# Autodesk Inventor assembly: standing_robot_ver.1
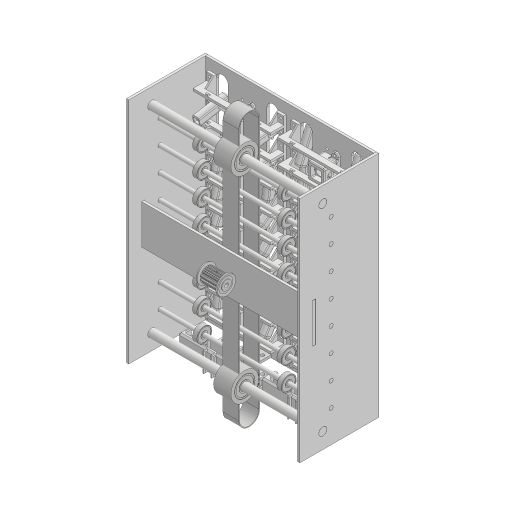
[picture p0: Inventor's stored thumbnail of the model, 512x512]
Saved by Autodesk Inventor 2024 (Build 280153000, 153)
## iProperties
Created: 2023-11-09
Part Number: standing_robot_ver.1
Document SubType Name: Assembly
Designer: moonshot
Author: moonshot
## Documents named in this file (18)
- C:\Users\moonshot\Desktop\ikisawa\ikisawa\experiment8_standing\standing_robot\standing_robot_ver.4.iam
- C:\Users\moonshot\Desktop\ikisawa\ikisawa\experiment8_standing\leg_unit\cover.ver1.ipt
- C:\Users\moonshot\Desktop\ikisawa\ikisawa\experiment8_standing\leg_unit\leg.ipt
- C:\Users\moonshot\Desktop\ikisawa\ikisawa\experiment8_standing\leg_unit\shaft_leg.ipt
- C:\Users\moonshot\Desktop\ikisawa\ikisawa\experiment8_standing\leg_unit\parent_ver.1.ipt
- C:\Users\moonshot\Desktop\ikisawa\ikisawa\experiment8_standing\floor\floor_ver.1.ipt
- C:\Users\moonshot\Desktop\ikisawa\ikisawa\experiment8_standing\belt\ATBT-720T5200-B-P30_info-1-16-16.ipt
- C:\Users\moonshot\Desktop\ikisawa\ikisawa\experiment8_standing\guide\guide_ver.2.ipt
- C:\Users\moonshot\Desktop\ikisawa\ikisawa\experiment8_standing\pulley\AIS2024\TTPS12T5200-A-P5.iam
- C:\Users\moonshot\Desktop\ikisawa\ikisawa\experiment8_standing\adapter\adapter_repulsive_force_ver.3.ipt
- C:\Users\moonshot\Desktop\ikisawa\ikisawa\experiment8_standing\wall\wall_ver.1.ipt
- C:\Users\moonshot\Desktop\ikisawa\ikisawa\experiment8_standing\bearing\C-SE635ZZ.ipt
- C:\Users\moonshot\Desktop\ikisawa\ikisawa\experiment8_standing\bearing\shaft_bearing\shaft_bearing.ipt
- C:\Users\moonshot\Desktop\ikisawa\ikisawa\experiment8_standing\stage\stage_ver.1.ipt
- C:\Users\moonshot\Desktop\ikisawa\ikisawa\experiment8_standing\idler\AIS2024\C-AFBD22-35W.iam
- C:\Users\moonshot\Desktop\ikisawa\ikisawa\experiment8_standing\bearing\shaft_bearing\shaft_idler_ver.1.ipt
- C:\Users\moonshot\Desktop\ikisawa\ikisawa\experiment8_standing\magnet\magnet_10-10-6.ipt
- C:\Users\moonshot\Desktop\ikisawa\ikisawa\experiment8_standing\magnet\magnet_holder_ver.1.ipt
## Components (146 placed, 17 different names)
1. floor_ver.1:1 — フラッシュ:3, フラッシュ:4, フラッシュ:5, メイト:8, メイト:9, メイト:10, メイト:16, メイト:17, メイト:18, メイト:4, メイト:5, メイト:15, メイト:14, メイト:19, メイト:20, メイト:21, メイト:40, フラッシュ:11, フラッシュ:12, メイト:55, メイト:56, メイト:60, メイト:61, メイト:62, メイト:63, メイト:67, メイト:68, メイト:69, メイト:70, メイト:71, メイト:72, メイト:73, メイト:74, メイト:75, メイト:79, メイト:80, メイト:81, メイト:82, メイト:83, メイト:87, メイト:88, メイト:89, メイト:90, メイト:91, メイト:95, メイト:96, メイト:97, メイト:98, メイト:99, メイト:103, メイト:104, メイト:105, メイト:106, メイト:107, メイト:111, メイト:112, メイト:113, メイト:114, メイト:115, メイト:119, メイト:120, メイト:121, メイト:122, メイト:123, メイト:127, メイト:128, メイト:129, メイト:130, メイト:131, メイト:135, メイト:136, メイト:137, メイト:138, メイト:139, メイト:143, メイト:144, メイト:145, メイト:146, メイト:147, メイト:151, メイト:152, メイト:153, メイト:154, メイト:155, メイト:159, メイト:160, メイト:161, メイト:162, メイト:163, メイト:164, メイト:165, メイト:166, メイト:167, メイト:168, メイト:169, メイト:170, メイト:171, メイト:172, メイト:173, メイト:174, メイト:175, メイト:176, メイト:177, メイト:178, メイト:179, メイト:180, メイト:181, メイト:182, メイト:183, メイト:184, メイト:185, メイト:186, メイト:187, メイト:188, メイト:189, メイト:190, メイト:191, メイト:192, メイト:193, メイト:194, メイト:195, メイト:196, メイト:197, メイト:198, メイト:199, メイト:200, メイト:201, メイト:202, メイト:203, メイト:204, メイト:205, メイト:206, メイト:207, メイト:208, メイト:209, メイト:210, メイト:211, メイト:212, メイト:213, メイト:214, メイト:255, フラッシュ:51, フラッシュ:52
2. ATBT-720T5200-B-P30_info-1-16-16:1 — メイト:6, フラッシュ:6, メイト:32, メイト:33, メイト:34, メイト:35
3. TTPS12T5200-A-P5:1 [sub-assembly] — メイト:29, フラッシュ:9, メイト:50
4. adapter_repulsive_force_ver.3:1 — メイト:30, メイト:31, メイト:32, メイト:33, メイト:34, メイト:36, メイト:268, フラッシュ:59, フラッシュ:60, メイト:269, メイト:270, フラッシュ:61, メイト:275, メイト:276
5. adapter_repulsive_force_ver.3:2 — メイト:30, メイト:31, メイト:35, メイト:271, フラッシュ:62, メイト:272, メイト:273, フラッシュ:63, メイト:274, フラッシュ:64, フラッシュ:65, メイト:277, メイト:278
6. wall_ver.1:2 — メイト:40, フラッシュ:11, フラッシュ:12, フラッシュ:13, メイト:46, フラッシュ:14, メイト:48, メイト:51, フラッシュ:43, メイト:217, フラッシュ:44, メイト:218, フラッシュ:45, メイト:219, フラッシュ:46, メイト:220, フラッシュ:47, メイト:221, メイト:222, メイト:223, フラッシュ:48, フラッシュ:49, フラッシュ:50, メイト:252
7. stage_ver.1:1 — メイト:44, メイト:45, メイト:50, メイト:51
8. C-AFBD22-35W:1 [sub-assembly] — メイト:47, メイト:49
9. shaft_idler_ver.1:1 — フラッシュ:14, メイト:48, メイト:49
10. shaft_idler_ver.1:2 — フラッシュ:50, メイト:252, メイト:254
11. C-AFBD22-35W:2 [sub-assembly] — メイト:253, メイト:254
12. wall_ver.1:3 — メイト:255, フラッシュ:51, フラッシュ:52
13. magnet_10-10-6:1 — メイト:256, メイト:257, フラッシュ:53, メイト:268, フラッシュ:59, メイト:275
14. magnet_10-10-6:2 — メイト:258, メイト:259, フラッシュ:54, メイト:269, メイト:276
15. magnet_10-10-6:3 — メイト:260, メイト:261, フラッシュ:55, メイト:270, フラッシュ:61
16. magnet_10-10-6:4 — メイト:262, メイト:263, フラッシュ:56, メイト:271, メイト:272, フラッシュ:65
17. magnet_10-10-6:5 — メイト:266, メイト:267, フラッシュ:58, メイト:274, メイト:277
18. magnet_10-10-6:6 — メイト:264, メイト:265, フラッシュ:57, メイト:273, メイト:278
19. magnet_holder_ver.1:1 — メイト:256, メイト:257, フラッシュ:53
20. magnet_holder_ver.1:2 — メイト:258, メイト:259, フラッシュ:54, フラッシュ:60
21. magnet_holder_ver.1:3 — メイト:260, メイト:261, フラッシュ:55
22. magnet_holder_ver.1:4 — メイト:262, メイト:263, フラッシュ:56, フラッシュ:62
23. magnet_holder_ver.1:5 — メイト:264, メイト:265, フラッシュ:57, フラッシュ:63
24. magnet_holder_ver.1:6 — メイト:266, メイト:267, フラッシュ:58, フラッシュ:64
25. cover.ver1:1 — フラッシュ:1, スライダ:1, メイト:8, メイト:9, メイト:10, メイト:36
26. leg:1 — メイト:2, メイト:5
27. leg:2 — メイト:3, メイト:4
28. shaft_leg:1 — メイト:1, フラッシュ:2, メイト:2, メイト:3
29. parent_ver.1:1 — フラッシュ:1, スライダ:1, メイト:1, フラッシュ:2, メイト:41
30. cover.ver1:2 — メイト:16, メイト:17, メイト:18
31. leg:3 — メイト:15, メイト:71
32. leg:4 — メイト:14
33. shaft_leg:2
34. parent_ver.1:2 — メイト:225
35. cover.ver1:3 — メイト:55, メイト:56, メイト:63
36. leg:5
37. leg:6 — メイト:70
38. shaft_leg:3
39. parent_ver.1:3 — メイト:231
40. cover.ver1:4 — メイト:60, メイト:61, メイト:62
41. leg:7 — メイト:73
42. leg:8 — メイト:72
43. shaft_leg:4
44. parent_ver.1:4 — メイト:234
45. cover.ver1:5 — メイト:67, メイト:68, メイト:69
46. leg:9 — メイト:74
47. leg:10 — メイト:75
48. shaft_leg:5
49. parent_ver.1:5 — メイト:239
50. cover.ver1:6 — メイト:79, メイト:80, メイト:81
51. leg:11 — メイト:83
52. leg:12 — メイト:82
53. shaft_leg:6
54. parent_ver.1:6 — メイト:243
55. cover.ver1:7 — メイト:87, メイト:88, メイト:89
56. leg:13 — メイト:90
57. leg:14 — メイト:91
58. shaft_leg:7
59. parent_ver.1:7 — メイト:247
60. cover.ver1:8 — メイト:95, メイト:96, メイト:97
61. leg:15 — メイト:98
62. leg:16 — メイト:99
63. shaft_leg:8
64. parent_ver.1:8 — メイト:251
65. cover.ver1:9 — メイト:103, メイト:104, メイト:105, メイト:216
66. leg:17 — メイト:106
67. leg:18 — メイト:107
68. shaft_leg:9
69. parent_ver.1:9
70. cover.ver1:10 — メイト:111, メイト:112, メイト:113
71. leg:19 — メイト:114
72. leg:20 — メイト:115
73. shaft_leg:10
74. parent_ver.1:10 — メイト:230
75. cover.ver1:11 — メイト:119, メイト:120, メイト:121
76. leg:21 — メイト:123
77. leg:22 — メイト:122
78. shaft_leg:11
79. parent_ver.1:11 — メイト:227
80. cover.ver1:12 — メイト:127, メイト:128, メイト:129
81. leg:23 — メイト:131
82. leg:24 — メイト:130
83. shaft_leg:12
84. parent_ver.1:12 — メイト:235
85. cover.ver1:13 — メイト:135, メイト:136, メイト:137
86. leg:25 — メイト:139
87. leg:26 — メイト:138
88. shaft_leg:13
89. parent_ver.1:13 — メイト:238
90. cover.ver1:14 — メイト:143, メイト:144, メイト:145
91. leg:27 — メイト:147
92. leg:28 — メイト:146
93. shaft_leg:14
94. parent_ver.1:14 — メイト:242
95. cover.ver1:15 — メイト:151, メイト:152, メイト:153
96. leg:29 — メイト:154
97. leg:30 — メイト:155
98. shaft_leg:15
99. parent_ver.1:15 — メイト:246
100. cover.ver1:16 — メイト:159, メイト:160, メイト:161
101. leg:31 — メイト:163
102. leg:32 — メイト:162
103. shaft_leg:16
104. parent_ver.1:16 — メイト:250
105. guide_ver.2:1 — メイト:19, メイト:20, メイト:21
106. guide_ver.2:2 — メイト:164, メイト:165, メイト:166
107. guide_ver.2:3 — メイト:167, メイト:168, メイト:169
108. guide_ver.2:4 — メイト:170, メイト:171, メイト:172
109. guide_ver.2:5 — メイト:173, メイト:174, メイト:175
110. guide_ver.2:6 — メイト:176, メイト:177, メイト:178
111. guide_ver.2:7 — メイト:179, メイト:180, メイト:181
112. guide_ver.2:8 — メイト:182, メイト:183, メイト:184
113. guide_ver.2:9 — メイト:185, メイト:186, メイト:187
114. guide_ver.2:10 — メイト:188, メイト:189, メイト:190
115. guide_ver.2:11 — メイト:191, メイト:192, メイト:193
116. guide_ver.2:12 — メイト:194, メイト:195, メイト:196
117. guide_ver.2:13 — メイト:197, メイト:198, メイト:199
118. guide_ver.2:14 — メイト:200, メイト:201, メイト:202
119. guide_ver.2:15 — メイト:203, メイト:204, メイト:205
120. guide_ver.2:16 — メイト:206, メイト:207, メイト:208
121. guide_ver.2:17 — メイト:209, メイト:210, メイト:211
122. guide_ver.2:18 — メイト:212, メイト:213, メイト:214
123. shaft_bearing:1 — フラッシュ:13, メイト:43, メイト:46, メイト:215
124. shaft_bearing:2 — フラッシュ:43, メイト:217, メイト:224, メイト:226
125. shaft_bearing:3 — フラッシュ:44, メイト:218, メイト:228, メイト:229
126. shaft_bearing:4 — フラッシュ:45, メイト:219, メイト:232, メイト:233
127. shaft_bearing:5 — フラッシュ:46, メイト:220, メイト:236, メイト:237
128. shaft_bearing:6 — フラッシュ:47, メイト:221, メイト:240, メイト:241
129. shaft_bearing:7 — メイト:222, フラッシュ:48, メイト:244, メイト:245
130. shaft_bearing:8 — メイト:223, フラッシュ:49, メイト:248, メイト:249
131. C-SE635ZZ:1 — メイト:41, メイト:43
132. C-SE635ZZ:2 — メイト:215, メイト:216
133. C-SE635ZZ:3 — メイト:224, メイト:225
134. C-SE635ZZ:4 — メイト:226, メイト:227
135. C-SE635ZZ:5 — メイト:228, メイト:231
136. C-SE635ZZ:6 — メイト:229, メイト:230
137. C-SE635ZZ:7 — メイト:232, メイト:234
138. C-SE635ZZ:8 — メイト:233, メイト:235
139. C-SE635ZZ:9 — メイト:236, メイト:239
140. C-SE635ZZ:10 — メイト:237, メイト:238
141. C-SE635ZZ:11 — メイト:240, メイト:243
142. C-SE635ZZ:12 — メイト:241, メイト:242
143. C-SE635ZZ:13 — メイト:244, メイト:247
144. C-SE635ZZ:14 — メイト:245, メイト:246
145. C-SE635ZZ:15 — メイト:248, メイト:251
146. C-SE635ZZ:16 — メイト:249, メイト:250
## Relationships (346: Mate 266, Flush 64, TranslationJoint 16)
- フラッシュ:1 [Flush]: cover.ver1:1 ↔ parent_ver.1:1
- スライダ:1 [TranslationJoint]: cover.ver1:1 ↔ parent_ver.1:1
- メイト:1 [Mate]: shaft_leg:1 ↔ parent_ver.1:1
- フラッシュ:2 [Flush]: shaft_leg:1 ↔ parent_ver.1:1
- メイト:2 [Mate]: leg:1 ↔ shaft_leg:1
- メイト:3 [Mate]: leg:2 ↔ shaft_leg:1
- メイト:4 [Mate] (2.5 mm): floor_ver.1:1 ↔ leg:2
- メイト:5 [Mate] (2.5 mm): floor_ver.1:1 ↔ leg:1
- フラッシュ:3 [Flush]: floor_ver.1:1
- フラッシュ:4 [Flush]: floor_ver.1:1
- フラッシュ:5 [Flush]: floor_ver.1:1
- メイト:6 [Mate]: ATBT-720T5200-B-P30_info-1-16-16:1
- フラッシュ:6 [Flush]: ATBT-720T5200-B-P30_info-1-16-16:1
- メイト:8 [Mate]: floor_ver.1:1 ↔ cover.ver1:1
- メイト:9 [Mate]: floor_ver.1:1 ↔ cover.ver1:1
- メイト:10 [Mate]: floor_ver.1:1 ↔ cover.ver1:1
- [Flush]: cover.ver1:2 ↔ parent_ver.1:2
- [TranslationJoint]: cover.ver1:2 ↔ parent_ver.1:2
- [Mate]: shaft_leg:2 ↔ parent_ver.1:2
- [Flush]: shaft_leg:2 ↔ parent_ver.1:2
- [Mate]: leg:3 ↔ shaft_leg:2
- [Mate]: leg:4 ↔ shaft_leg:2
- メイト:14 [Mate] (2.5 mm): floor_ver.1:1 ↔ leg:4
- メイト:15 [Mate] (2.5 mm): floor_ver.1:1 ↔ leg:3
- メイト:16 [Mate]: floor_ver.1:1 ↔ cover.ver1:2
- メイト:17 [Mate]: floor_ver.1:1 ↔ cover.ver1:2
- メイト:18 [Mate]: floor_ver.1:1 ↔ cover.ver1:2
- メイト:19 [Mate]: floor_ver.1:1 ↔ guide_ver.2:1
- メイト:20 [Mate]: floor_ver.1:1 ↔ guide_ver.2:1
- メイト:21 [Mate]: floor_ver.1:1 ↔ guide_ver.2:1
- メイト:29 [Mate]: TTPS12T5200-A-P5:1
- フラッシュ:9 [Flush]: TTPS12T5200-A-P5:1
- メイト:50 [Mate] (13 mm): TTPS12T5200-A-P5:1 ↔ stage_ver.1:1
- メイト:30 [Mate]: adapter_repulsive_force_ver.3:1 ↔ adapter_repulsive_force_ver.3:2
- メイト:31 [Mate]: adapter_repulsive_force_ver.3:1 ↔ adapter_repulsive_force_ver.3:2
- メイト:32 [Mate]: ATBT-720T5200-B-P30_info-1-16-16:1 ↔ adapter_repulsive_force_ver.3:1
- メイト:33 [Mate]: ATBT-720T5200-B-P30_info-1-16-16:1 ↔ adapter_repulsive_force_ver.3:1
- メイト:34 [Mate]: ATBT-720T5200-B-P30_info-1-16-16:1 ↔ adapter_repulsive_force_ver.3:1
- メイト:35 [Mate]: ATBT-720T5200-B-P30_info-1-16-16:1 ↔ adapter_repulsive_force_ver.3:2
- メイト:36 [Mate] (1 mm): adapter_repulsive_force_ver.3:1 ↔ cover.ver1:1
- メイト:40 [Mate]: floor_ver.1:1 ↔ wall_ver.1:2
- フラッシュ:11 [Flush]: floor_ver.1:1 ↔ wall_ver.1:2
- フラッシュ:12 [Flush]: floor_ver.1:1 ↔ wall_ver.1:2
- メイト:41 [Mate]: parent_ver.1:1 ↔ C-SE635ZZ:1
- フラッシュ:13 [Flush]: wall_ver.1:2 ↔ shaft_bearing:1
- メイト:43 [Mate]: shaft_bearing:1 ↔ C-SE635ZZ:1
- メイト:44 [Mate]: stage_ver.1:1
- メイト:45 [Mate]: stage_ver.1:1
- メイト:46 [Mate]: wall_ver.1:2 ↔ shaft_bearing:1
- メイト:47 [Mate]: C-AFBD22-35W:1
- フラッシュ:14 [Flush]: wall_ver.1:2 ↔ shaft_idler_ver.1:1
- メイト:48 [Mate]: wall_ver.1:2 ↔ shaft_idler_ver.1:1
- メイト:49 [Mate]: C-AFBD22-35W:1 ↔ shaft_idler_ver.1:1
- メイト:51 [Mate] (20 mm): wall_ver.1:2 ↔ stage_ver.1:1
- [Flush]: cover.ver1:3 ↔ parent_ver.1:3
- [TranslationJoint]: cover.ver1:3 ↔ parent_ver.1:3
- [Mate]: shaft_leg:3 ↔ parent_ver.1:3
- [Flush]: shaft_leg:3 ↔ parent_ver.1:3
- [Mate]: leg:5 ↔ shaft_leg:3
- [Mate]: leg:6 ↔ shaft_leg:3
- メイト:55 [Mate]: floor_ver.1:1 ↔ cover.ver1:3
- メイト:56 [Mate]: floor_ver.1:1 ↔ cover.ver1:3
- [Flush]: cover.ver1:4 ↔ parent_ver.1:4
- [TranslationJoint]: cover.ver1:4 ↔ parent_ver.1:4
- [Mate]: shaft_leg:4 ↔ parent_ver.1:4
- [Flush]: shaft_leg:4 ↔ parent_ver.1:4
- [Mate]: leg:7 ↔ shaft_leg:4
- [Mate]: leg:8 ↔ shaft_leg:4
- メイト:60 [Mate]: floor_ver.1:1 ↔ cover.ver1:4
- メイト:61 [Mate]: floor_ver.1:1 ↔ cover.ver1:4
- メイト:62 [Mate]: floor_ver.1:1 ↔ cover.ver1:4
- メイト:63 [Mate]: floor_ver.1:1 ↔ cover.ver1:3
- [Flush]: cover.ver1:5 ↔ parent_ver.1:5
- [TranslationJoint]: cover.ver1:5 ↔ parent_ver.1:5
- [Mate]: shaft_leg:5 ↔ parent_ver.1:5
- [Flush]: shaft_leg:5 ↔ parent_ver.1:5
- [Mate]: leg:9 ↔ shaft_leg:5
- [Mate]: leg:10 ↔ shaft_leg:5
- メイト:67 [Mate]: floor_ver.1:1 ↔ cover.ver1:5
- メイト:68 [Mate]: floor_ver.1:1 ↔ cover.ver1:5
- メイト:69 [Mate]: floor_ver.1:1 ↔ cover.ver1:5
- メイト:70 [Mate] (2.5 mm): floor_ver.1:1 ↔ leg:6
- メイト:71 [Mate] (2.5 mm): floor_ver.1:1 ↔ leg:3
- メイト:72 [Mate] (2.5 mm): floor_ver.1:1 ↔ leg:8
- メイト:73 [Mate] (2.5 mm): floor_ver.1:1 ↔ leg:7
- メイト:74 [Mate] (2.5 mm): floor_ver.1:1 ↔ leg:9
- メイト:75 [Mate] (2.5 mm): floor_ver.1:1 ↔ leg:10
- [Flush]: cover.ver1:6 ↔ parent_ver.1:6
- [TranslationJoint]: cover.ver1:6 ↔ parent_ver.1:6
- [Mate]: shaft_leg:6 ↔ parent_ver.1:6
- [Flush]: shaft_leg:6 ↔ parent_ver.1:6
- [Mate]: leg:11 ↔ shaft_leg:6
- [Mate]: leg:12 ↔ shaft_leg:6
- メイト:79 [Mate]: floor_ver.1:1 ↔ cover.ver1:6
- メイト:80 [Mate]: floor_ver.1:1 ↔ cover.ver1:6
- メイト:81 [Mate]: floor_ver.1:1 ↔ cover.ver1:6
- メイト:82 [Mate] (2.5 mm): floor_ver.1:1 ↔ leg:12
- メイト:83 [Mate] (2.5 mm): floor_ver.1:1 ↔ leg:11
- [Flush]: cover.ver1:7 ↔ parent_ver.1:7
- [TranslationJoint]: cover.ver1:7 ↔ parent_ver.1:7
- [Mate]: shaft_leg:7 ↔ parent_ver.1:7
- [Flush]: shaft_leg:7 ↔ parent_ver.1:7
- [Mate]: leg:13 ↔ shaft_leg:7
- [Mate]: leg:14 ↔ shaft_leg:7
- メイト:87 [Mate]: floor_ver.1:1 ↔ cover.ver1:7
- メイト:88 [Mate]: floor_ver.1:1 ↔ cover.ver1:7
- メイト:89 [Mate]: floor_ver.1:1 ↔ cover.ver1:7
- メイト:90 [Mate] (2.5 mm): floor_ver.1:1 ↔ leg:13
- メイト:91 [Mate] (2.5 mm): floor_ver.1:1 ↔ leg:14
- [Flush]: cover.ver1:8 ↔ parent_ver.1:8
- [TranslationJoint]: cover.ver1:8 ↔ parent_ver.1:8
- [Mate]: shaft_leg:8 ↔ parent_ver.1:8
- [Flush]: shaft_leg:8 ↔ parent_ver.1:8
- [Mate]: leg:15 ↔ shaft_leg:8
- [Mate]: leg:16 ↔ shaft_leg:8
- メイト:95 [Mate]: floor_ver.1:1 ↔ cover.ver1:8
- メイト:96 [Mate]: floor_ver.1:1 ↔ cover.ver1:8
- メイト:97 [Mate]: floor_ver.1:1 ↔ cover.ver1:8
- メイト:98 [Mate] (2.5 mm): floor_ver.1:1 ↔ leg:15
- メイト:99 [Mate] (2.5 mm): floor_ver.1:1 ↔ leg:16
- [Flush]: cover.ver1:9 ↔ parent_ver.1:9
- [TranslationJoint]: cover.ver1:9 ↔ parent_ver.1:9
- [Mate]: shaft_leg:9 ↔ parent_ver.1:9
- [Flush]: shaft_leg:9 ↔ parent_ver.1:9
- [Mate]: leg:17 ↔ shaft_leg:9
- [Mate]: leg:18 ↔ shaft_leg:9
- メイト:103 [Mate]: floor_ver.1:1 ↔ cover.ver1:9
- メイト:104 [Mate]: floor_ver.1:1 ↔ cover.ver1:9
- メイト:105 [Mate]: floor_ver.1:1 ↔ cover.ver1:9
- メイト:106 [Mate] (2.5 mm): floor_ver.1:1 ↔ leg:17
- メイト:107 [Mate] (2.5 mm): floor_ver.1:1 ↔ leg:18
- [Flush]: cover.ver1:10 ↔ parent_ver.1:10
- [TranslationJoint]: cover.ver1:10 ↔ parent_ver.1:10
- [Mate]: shaft_leg:10 ↔ parent_ver.1:10
- [Flush]: shaft_leg:10 ↔ parent_ver.1:10
- [Mate]: leg:19 ↔ shaft_leg:10
- [Mate]: leg:20 ↔ shaft_leg:10
- メイト:111 [Mate]: floor_ver.1:1 ↔ cover.ver1:10
- メイト:112 [Mate]: floor_ver.1:1 ↔ cover.ver1:10
- メイト:113 [Mate]: floor_ver.1:1 ↔ cover.ver1:10
- メイト:114 [Mate] (2.5 mm): floor_ver.1:1 ↔ leg:19
- メイト:115 [Mate] (2.5 mm): floor_ver.1:1 ↔ leg:20
- [Flush]: cover.ver1:11 ↔ parent_ver.1:11
- [TranslationJoint]: cover.ver1:11 ↔ parent_ver.1:11
- [Mate]: shaft_leg:11 ↔ parent_ver.1:11
- [Flush]: shaft_leg:11 ↔ parent_ver.1:11
- [Mate]: leg:21 ↔ shaft_leg:11
- [Mate]: leg:22 ↔ shaft_leg:11
- メイト:119 [Mate]: floor_ver.1:1 ↔ cover.ver1:11
- メイト:120 [Mate]: floor_ver.1:1 ↔ cover.ver1:11
- メイト:121 [Mate]: floor_ver.1:1 ↔ cover.ver1:11
- メイト:122 [Mate] (2.5 mm): floor_ver.1:1 ↔ leg:22
- メイト:123 [Mate] (2.5 mm): floor_ver.1:1 ↔ leg:21
- [Flush]: cover.ver1:12 ↔ parent_ver.1:12
- [TranslationJoint]: cover.ver1:12 ↔ parent_ver.1:12
- [Mate]: shaft_leg:12 ↔ parent_ver.1:12
- [Flush]: shaft_leg:12 ↔ parent_ver.1:12
- [Mate]: leg:23 ↔ shaft_leg:12
- [Mate]: leg:24 ↔ shaft_leg:12
- メイト:127 [Mate]: floor_ver.1:1 ↔ cover.ver1:12
- メイト:128 [Mate]: floor_ver.1:1 ↔ cover.ver1:12
- メイト:129 [Mate]: floor_ver.1:1 ↔ cover.ver1:12
- メイト:130 [Mate] (2.5 mm): floor_ver.1:1 ↔ leg:24
- メイト:131 [Mate] (2.5 mm): floor_ver.1:1 ↔ leg:23
- [Flush]: cover.ver1:13 ↔ parent_ver.1:13
- [TranslationJoint]: cover.ver1:13 ↔ parent_ver.1:13
- [Mate]: shaft_leg:13 ↔ parent_ver.1:13
- [Flush]: shaft_leg:13 ↔ parent_ver.1:13
- [Mate]: leg:25 ↔ shaft_leg:13
- [Mate]: leg:26 ↔ shaft_leg:13
- メイト:135 [Mate]: floor_ver.1:1 ↔ cover.ver1:13
- メイト:136 [Mate]: floor_ver.1:1 ↔ cover.ver1:13
- メイト:137 [Mate]: floor_ver.1:1 ↔ cover.ver1:13
- メイト:138 [Mate] (2.5 mm): floor_ver.1:1 ↔ leg:26
- メイト:139 [Mate] (2.5 mm): floor_ver.1:1 ↔ leg:25
- [Flush]: cover.ver1:14 ↔ parent_ver.1:14
- [TranslationJoint]: cover.ver1:14 ↔ parent_ver.1:14
- [Mate]: shaft_leg:14 ↔ parent_ver.1:14
- [Flush]: shaft_leg:14 ↔ parent_ver.1:14
- [Mate]: leg:27 ↔ shaft_leg:14
- [Mate]: leg:28 ↔ shaft_leg:14
- メイト:143 [Mate]: floor_ver.1:1 ↔ cover.ver1:14
- メイト:144 [Mate]: floor_ver.1:1 ↔ cover.ver1:14
- メイト:145 [Mate]: floor_ver.1:1 ↔ cover.ver1:14
- メイト:146 [Mate] (2.5 mm): floor_ver.1:1 ↔ leg:28
- メイト:147 [Mate] (2.5 mm): floor_ver.1:1 ↔ leg:27
- [Flush]: cover.ver1:15 ↔ parent_ver.1:15
- [TranslationJoint]: cover.ver1:15 ↔ parent_ver.1:15
- [Mate]: shaft_leg:15 ↔ parent_ver.1:15
- [Flush]: shaft_leg:15 ↔ parent_ver.1:15
- [Mate]: leg:29 ↔ shaft_leg:15
- [Mate]: leg:30 ↔ shaft_leg:15
- メイト:151 [Mate]: floor_ver.1:1 ↔ cover.ver1:15
- メイト:152 [Mate]: floor_ver.1:1 ↔ cover.ver1:15
- メイト:153 [Mate]: floor_ver.1:1 ↔ cover.ver1:15
- メイト:154 [Mate] (2.5 mm): floor_ver.1:1 ↔ leg:29
- メイト:155 [Mate] (2.5 mm): floor_ver.1:1 ↔ leg:30
- [Flush]: cover.ver1:16 ↔ parent_ver.1:16
- [TranslationJoint]: cover.ver1:16 ↔ parent_ver.1:16
- [Mate]: shaft_leg:16 ↔ parent_ver.1:16
- [Flush]: shaft_leg:16 ↔ parent_ver.1:16
- [Mate]: leg:31 ↔ shaft_leg:16
- [Mate]: leg:32 ↔ shaft_leg:16
- メイト:159 [Mate]: floor_ver.1:1 ↔ cover.ver1:16
- メイト:160 [Mate]: floor_ver.1:1 ↔ cover.ver1:16
- メイト:161 [Mate]: floor_ver.1:1 ↔ cover.ver1:16
- メイト:162 [Mate] (2.5 mm): floor_ver.1:1 ↔ leg:32
- メイト:163 [Mate] (2.5 mm): floor_ver.1:1 ↔ leg:31
- メイト:164 [Mate]: floor_ver.1:1 ↔ guide_ver.2:2
- メイト:165 [Mate]: floor_ver.1:1 ↔ guide_ver.2:2
- メイト:166 [Mate]: floor_ver.1:1 ↔ guide_ver.2:2
- メイト:167 [Mate]: floor_ver.1:1 ↔ guide_ver.2:3
- メイト:168 [Mate]: floor_ver.1:1 ↔ guide_ver.2:3
- メイト:169 [Mate]: floor_ver.1:1 ↔ guide_ver.2:3
- メイト:170 [Mate]: floor_ver.1:1 ↔ guide_ver.2:4
- メイト:171 [Mate]: floor_ver.1:1 ↔ guide_ver.2:4
- メイト:172 [Mate]: floor_ver.1:1 ↔ guide_ver.2:4
- メイト:173 [Mate]: floor_ver.1:1 ↔ guide_ver.2:5
- メイト:174 [Mate]: floor_ver.1:1 ↔ guide_ver.2:5
- メイト:175 [Mate]: floor_ver.1:1 ↔ guide_ver.2:5
- メイト:176 [Mate]: floor_ver.1:1 ↔ guide_ver.2:6
- メイト:177 [Mate]: floor_ver.1:1 ↔ guide_ver.2:6
- メイト:178 [Mate]: floor_ver.1:1 ↔ guide_ver.2:6
- メイト:179 [Mate]: floor_ver.1:1 ↔ guide_ver.2:7
- メイト:180 [Mate]: floor_ver.1:1 ↔ guide_ver.2:7
- メイト:181 [Mate]: floor_ver.1:1 ↔ guide_ver.2:7
- メイト:182 [Mate]: floor_ver.1:1 ↔ guide_ver.2:8
- メイト:183 [Mate]: floor_ver.1:1 ↔ guide_ver.2:8
- メイト:184 [Mate]: floor_ver.1:1 ↔ guide_ver.2:8
- メイト:185 [Mate]: floor_ver.1:1 ↔ guide_ver.2:9
- メイト:186 [Mate]: floor_ver.1:1 ↔ guide_ver.2:9
- メイト:187 [Mate]: floor_ver.1:1 ↔ guide_ver.2:9
- メイト:188 [Mate]: floor_ver.1:1 ↔ guide_ver.2:10
- メイト:189 [Mate]: floor_ver.1:1 ↔ guide_ver.2:10
- メイト:190 [Mate]: floor_ver.1:1 ↔ guide_ver.2:10
- メイト:191 [Mate]: floor_ver.1:1 ↔ guide_ver.2:11
- メイト:192 [Mate]: floor_ver.1:1 ↔ guide_ver.2:11
- メイト:193 [Mate]: floor_ver.1:1 ↔ guide_ver.2:11
- メイト:194 [Mate]: floor_ver.1:1 ↔ guide_ver.2:12
- メイト:195 [Mate]: floor_ver.1:1 ↔ guide_ver.2:12
- メイト:196 [Mate]: floor_ver.1:1 ↔ guide_ver.2:12
- メイト:197 [Mate]: floor_ver.1:1 ↔ guide_ver.2:13
- メイト:198 [Mate]: floor_ver.1:1 ↔ guide_ver.2:13
- メイト:199 [Mate]: floor_ver.1:1 ↔ guide_ver.2:13
- メイト:200 [Mate]: floor_ver.1:1 ↔ guide_ver.2:14
- メイト:201 [Mate]: floor_ver.1:1 ↔ guide_ver.2:14
- メイト:202 [Mate]: floor_ver.1:1 ↔ guide_ver.2:14
- メイト:203 [Mate]: floor_ver.1:1 ↔ guide_ver.2:15
- メイト:204 [Mate]: floor_ver.1:1 ↔ guide_ver.2:15
- メイト:205 [Mate]: floor_ver.1:1 ↔ guide_ver.2:15
- メイト:206 [Mate]: floor_ver.1:1 ↔ guide_ver.2:16
- メイト:207 [Mate]: floor_ver.1:1 ↔ guide_ver.2:16
- メイト:208 [Mate]: floor_ver.1:1 ↔ guide_ver.2:16
- メイト:209 [Mate]: floor_ver.1:1 ↔ guide_ver.2:17
- メイト:210 [Mate]: floor_ver.1:1 ↔ guide_ver.2:17
- メイト:211 [Mate]: floor_ver.1:1 ↔ guide_ver.2:17
- メイト:212 [Mate]: floor_ver.1:1 ↔ guide_ver.2:18
- メイト:213 [Mate]: floor_ver.1:1 ↔ guide_ver.2:18
- メイト:214 [Mate]: floor_ver.1:1 ↔ guide_ver.2:18
- メイト:215 [Mate]: shaft_bearing:1 ↔ C-SE635ZZ:2
- メイト:216 [Mate]: cover.ver1:9 ↔ C-SE635ZZ:2
- フラッシュ:43 [Flush]: wall_ver.1:2 ↔ shaft_bearing:2
- メイト:217 [Mate]: wall_ver.1:2 ↔ shaft_bearing:2
- フラッシュ:44 [Flush]: wall_ver.1:2 ↔ shaft_bearing:3
- メイト:218 [Mate]: wall_ver.1:2 ↔ shaft_bearing:3
- フラッシュ:45 [Flush]: wall_ver.1:2 ↔ shaft_bearing:4
- メイト:219 [Mate]: wall_ver.1:2 ↔ shaft_bearing:4
- フラッシュ:46 [Flush]: wall_ver.1:2 ↔ shaft_bearing:5
- メイト:220 [Mate]: wall_ver.1:2 ↔ shaft_bearing:5
- フラッシュ:47 [Flush]: wall_ver.1:2 ↔ shaft_bearing:6
- メイト:221 [Mate]: wall_ver.1:2 ↔ shaft_bearing:6
- メイト:222 [Mate]: wall_ver.1:2 ↔ shaft_bearing:7
- メイト:223 [Mate]: wall_ver.1:2 ↔ shaft_bearing:8
- フラッシュ:48 [Flush]: wall_ver.1:2 ↔ shaft_bearing:7
- フラッシュ:49 [Flush]: wall_ver.1:2 ↔ shaft_bearing:8
- メイト:224 [Mate]: shaft_bearing:2 ↔ C-SE635ZZ:3
- メイト:225 [Mate]: parent_ver.1:2 ↔ C-SE635ZZ:3
- メイト:226 [Mate]: shaft_bearing:2 ↔ C-SE635ZZ:4
- メイト:227 [Mate]: parent_ver.1:11 ↔ C-SE635ZZ:4
- メイト:228 [Mate]: shaft_bearing:3 ↔ C-SE635ZZ:5
- メイト:229 [Mate]: shaft_bearing:3 ↔ C-SE635ZZ:6
- メイト:230 [Mate]: parent_ver.1:10 ↔ C-SE635ZZ:6
- メイト:231 [Mate]: parent_ver.1:3 ↔ C-SE635ZZ:5
- メイト:232 [Mate]: shaft_bearing:4 ↔ C-SE635ZZ:7
- メイト:233 [Mate]: shaft_bearing:4 ↔ C-SE635ZZ:8
- メイト:234 [Mate]: parent_ver.1:4 ↔ C-SE635ZZ:7
- メイト:235 [Mate]: parent_ver.1:12 ↔ C-SE635ZZ:8
- メイト:236 [Mate]: shaft_bearing:5 ↔ C-SE635ZZ:9
- メイト:237 [Mate]: shaft_bearing:5 ↔ C-SE635ZZ:10
- メイト:238 [Mate]: parent_ver.1:13 ↔ C-SE635ZZ:10
- メイト:239 [Mate]: parent_ver.1:5 ↔ C-SE635ZZ:9
- メイト:240 [Mate]: shaft_bearing:6 ↔ C-SE635ZZ:11
- メイト:241 [Mate]: shaft_bearing:6 ↔ C-SE635ZZ:12
- メイト:242 [Mate]: parent_ver.1:14 ↔ C-SE635ZZ:12
- メイト:243 [Mate]: parent_ver.1:6 ↔ C-SE635ZZ:11
- メイト:244 [Mate]: shaft_bearing:7 ↔ C-SE635ZZ:13
- メイト:245 [Mate]: shaft_bearing:7 ↔ C-SE635ZZ:14
- メイト:246 [Mate]: parent_ver.1:15 ↔ C-SE635ZZ:14
- メイト:247 [Mate]: parent_ver.1:7 ↔ C-SE635ZZ:13
- メイト:248 [Mate]: shaft_bearing:8 ↔ C-SE635ZZ:15
- メイト:249 [Mate]: shaft_bearing:8 ↔ C-SE635ZZ:16
- メイト:250 [Mate]: parent_ver.1:16 ↔ C-SE635ZZ:16
- メイト:251 [Mate]: parent_ver.1:8 ↔ C-SE635ZZ:15
- フラッシュ:50 [Flush]: wall_ver.1:2 ↔ shaft_idler_ver.1:2
- メイト:252 [Mate]: wall_ver.1:2 ↔ shaft_idler_ver.1:2
- メイト:253 [Mate]: C-AFBD22-35W:2
- メイト:254 [Mate]: shaft_idler_ver.1:2 ↔ C-AFBD22-35W:2
- メイト:255 [Mate]: floor_ver.1:1 ↔ wall_ver.1:3
- フラッシュ:51 [Flush]: floor_ver.1:1 ↔ wall_ver.1:3
- フラッシュ:52 [Flush]: floor_ver.1:1 ↔ wall_ver.1:3
- メイト:256 [Mate]: magnet_10-10-6:1 ↔ magnet_holder_ver.1:1
- メイト:257 [Mate]: magnet_10-10-6:1 ↔ magnet_holder_ver.1:1
- フラッシュ:53 [Flush]: magnet_10-10-6:1 ↔ magnet_holder_ver.1:1
- メイト:258 [Mate]: magnet_10-10-6:2 ↔ magnet_holder_ver.1:2
- メイト:259 [Mate]: magnet_10-10-6:2 ↔ magnet_holder_ver.1:2
- フラッシュ:54 [Flush]: magnet_10-10-6:2 ↔ magnet_holder_ver.1:2
- メイト:260 [Mate]: magnet_10-10-6:3 ↔ magnet_holder_ver.1:3
- メイト:261 [Mate]: magnet_10-10-6:3 ↔ magnet_holder_ver.1:3
- フラッシュ:55 [Flush]: magnet_10-10-6:3 ↔ magnet_holder_ver.1:3
- メイト:262 [Mate]: magnet_10-10-6:4 ↔ magnet_holder_ver.1:4
- メイト:263 [Mate]: magnet_10-10-6:4 ↔ magnet_holder_ver.1:4
- フラッシュ:56 [Flush]: magnet_10-10-6:4 ↔ magnet_holder_ver.1:4
- メイト:264 [Mate]: magnet_10-10-6:6 ↔ magnet_holder_ver.1:5
- メイト:265 [Mate]: magnet_10-10-6:6 ↔ magnet_holder_ver.1:5
- フラッシュ:57 [Flush]: magnet_10-10-6:6 ↔ magnet_holder_ver.1:5
- メイト:266 [Mate]: magnet_10-10-6:5 ↔ magnet_holder_ver.1:6
- メイト:267 [Mate]: magnet_10-10-6:5 ↔ magnet_holder_ver.1:6
- フラッシュ:58 [Flush]: magnet_10-10-6:5 ↔ magnet_holder_ver.1:6
- メイト:268 [Mate]: adapter_repulsive_force_ver.3:1 ↔ magnet_10-10-6:1
- フラッシュ:59 [Flush]: adapter_repulsive_force_ver.3:1 ↔ magnet_10-10-6:1
- フラッシュ:60 [Flush]: adapter_repulsive_force_ver.3:1 ↔ magnet_holder_ver.1:2
- メイト:269 [Mate]: adapter_repulsive_force_ver.3:1 ↔ magnet_10-10-6:2
- メイト:270 [Mate]: adapter_repulsive_force_ver.3:1 ↔ magnet_10-10-6:3
- フラッシュ:61 [Flush]: adapter_repulsive_force_ver.3:1 ↔ magnet_10-10-6:3
- メイト:271 [Mate]: adapter_repulsive_force_ver.3:2 ↔ magnet_10-10-6:4
- フラッシュ:62 [Flush]: adapter_repulsive_force_ver.3:2 ↔ magnet_holder_ver.1:4
- メイト:272 [Mate]: adapter_repulsive_force_ver.3:2 ↔ magnet_10-10-6:4
- メイト:273 [Mate]: adapter_repulsive_force_ver.3:2 ↔ magnet_10-10-6:6
- フラッシュ:63 [Flush]: adapter_repulsive_force_ver.3:2 ↔ magnet_holder_ver.1:5
- メイト:274 [Mate]: adapter_repulsive_force_ver.3:2 ↔ magnet_10-10-6:5
- フラッシュ:64 [Flush]: adapter_repulsive_force_ver.3:2 ↔ magnet_holder_ver.1:6
- メイト:275 [Mate]: adapter_repulsive_force_ver.3:1 ↔ magnet_10-10-6:1
- メイト:276 [Mate]: adapter_repulsive_force_ver.3:1 ↔ magnet_10-10-6:2
- フラッシュ:65 [Flush]: adapter_repulsive_force_ver.3:2 ↔ magnet_10-10-6:4
- メイト:277 [Mate]: adapter_repulsive_force_ver.3:2 ↔ magnet_10-10-6:5
- メイト:278 [Mate]: adapter_repulsive_force_ver.3:2 ↔ magnet_10-10-6:6
## Named parameters: d21_d1 = 0 mm, d22_d2 = 0 mm, d23_d3 = 2 mm, d24_d4 = 1.53773 mm, d25_d5 = -3 mm, d26_d6 = 0 mm, d27_d7 = 0 mm, d28_d8 = 0 mm, d29_d9 = 0 mm, d30_d10 = 2.5 mm, d31_d11 = 2.5 mm, d85_d6 = 0 mm, d86_d7 = 0 mm, d87_d8 = 0 mm, d88_d9 = 0 mm, d89_d1 = 0 mm, d90_d2 = 0 mm, d91_d3 = 2 mm, d92_d4 = 2 mm, d93_d5 = -3 mm, d96_d6 = 0 mm, d97_d7 = 0 mm, d98_d8 = 0 mm, d99_d9 = 0 mm, d100_d1 = 0 mm, d101_d2 = 0 mm, d102_d3 = 2 mm, d103_d4 = 2 mm, d104_d5 = -3 mm, d109_d6 = 0 mm, d110_d7 = 0 mm, d111_d8 = 0 mm, d112_d9 = 0 mm, d113_d1 = 0 mm, d114_d2 = 0 mm, d115_d3 = 2 mm, d116_d4 = 2 mm, d117_d5 = -3 mm, d127_d6 = 0 mm, d128_d7 = 0 mm, d129_d8 = 0 mm, d130_d9 = 0 mm, d131_d1 = 0 mm, d132_d2 = 0 mm, d133_d3 = 2 mm, d134_d4 = 2 mm, d135_d5 = -3 mm, d141_d6 = 0 mm, d142_d7 = 0 mm, d143_d8 = 0 mm, d144_d9 = 0 mm, d145_d1 = 0 mm, d146_d2 = 0 mm, d147_d3 = 2 mm, d148_d4 = 2 mm, d149_d5 = -3 mm, d155_d6 = 0 mm, d156_d7 = 0 mm, d157_d8 = 0 mm, d158_d9 = 0 mm, d159_d1 = 0 mm, d160_d2 = 0 mm, d161_d3 = 2 mm, d162_d4 = 2 mm, d163_d5 = -3 mm, d169_d6 = 0 mm, d170_d7 = 0 mm, d171_d8 = 0 mm, d172_d9 = 0 mm, d173_d1 = 0 mm, d174_d2 = 0 mm, d175_d3 = 2 mm, d176_d4 = 2 mm, d177_d5 = -3 mm, d183_d6 = 0 mm, d184_d7 = 0 mm, d185_d8 = 0 mm, d186_d9 = 0 mm, d187_d1 = 0 mm, d188_d2 = 0 mm, d189_d3 = 2 mm, d190_d4 = -3 mm, d191_d5 = -3 mm, d197_d6 = 0 mm, d198_d7 = 0 mm, d199_d8 = 0 mm, d200_d9 = 0 mm, d201_d1 = 0 mm, d202_d2 = 0 mm, d203_d3 = 2 mm, d204_d4 = 0.93544 mm, d205_d5 = -3 mm, d211_d6 = 0 mm, d212_d7 = 0 mm, d213_d8 = 0 mm, d214_d9 = 0 mm, d215_d1 = 0 mm, d216_d2 = 0 mm, d217_d3 = 2 mm, d218_d4 = 2 mm, d219_d5 = -3 mm, d225_d6 = 0 mm, d226_d7 = 0 mm, d227_d8 = 0 mm, d228_d9 = 0 mm, d229_d1 = 0 mm, d230_d2 = 0 mm, d231_d3 = 2 mm, d232_d4 = 1.0893 mm, d233_d5 = -3 mm, d239_d6 = 0 mm, d240_d7 = 0 mm, d241_d8 = 0 mm, d242_d9 = 0 mm, d243_d1 = 0 mm, d244_d2 = 0 mm, d245_d3 = 2 mm, d246_d4 = 2 mm, d247_d5 = -3 mm, d253_d6 = 0 mm, d254_d7 = 0 mm, d255_d8 = 0 mm, d256_d9 = 0 mm, d257_d1 = 0 mm, d258_d2 = 0 mm, d259_d3 = 2 mm, d260_d4 = -0.95451 mm, d261_d5 = -3 mm, d267_d6 = 0 mm, d268_d7 = 0 mm, d269_d8 = 0 mm, d270_d9 = 0 mm, d271_d1 = 0 mm, d272_d2 = 0 mm, d273_d3 = 2 mm, d274_d4 = -2.99584 mm, d275_d5 = -3 mm
